# Autodesk Inventor assembly: SPE48V1 Roldana Acrilico
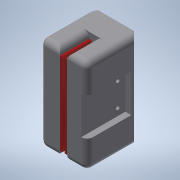
[picture p0: Inventor's stored thumbnail of the model, 180x180]
Saved by Autodesk Inventor 2021.2 (Build 252289000, 289)
## iProperties
Created: 2026-09-01
Part Number: SPE48V1 Roldana Acrilico
Document SubType Name: Assembly
Designer: nelso
Author: nelso
## Documents named in this file (3)
- C:\Users\nelso\Desktop\Soporte-Paciente-Espinografia\Workspace\SPE48V1 Roldana Acrilico.iam
- C:\Users\nelso\Desktop\Soporte-Paciente-Espinografia\Workspace\SP45V1 Plastico Roldana.ipt
- C:\Users\nelso\Desktop\Soporte-Paciente-Espinografia\Workspace\SP46V1 Felpa Roldana.ipt
## Components (3 placed, 2 different names)
1. SP45V1 Plastico Roldana:1 — Mate:1, Mate:2, Flush:1, Flush:2, Flush:3, Mate:3
2. SP46V1 Felpa Roldana:1 — Mate:1, Flush:1, Flush:3
3. SP46V1 Felpa Roldana:2 — Mate:2, Flush:2, Mate:3
## Relationships (6: Mate 3, Flush 3)
- Mate:1: SP45V1 Plastico Roldana:1 ↔ SP46V1 Felpa Roldana:1
- Mate:2: SP45V1 Plastico Roldana:1 ↔ SP46V1 Felpa Roldana:2
- Flush:1: SP45V1 Plastico Roldana:1 ↔ SP46V1 Felpa Roldana:1
- Flush:2: SP45V1 Plastico Roldana:1 ↔ SP46V1 Felpa Roldana:2
- Flush:3: SP45V1 Plastico Roldana:1 ↔ SP46V1 Felpa Roldana:1
- Mate:3: SP45V1 Plastico Roldana:1 ↔ SP46V1 Felpa Roldana:2
